# Autodesk Inventor assembly: tortoise
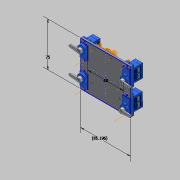
[picture p0: Inventor's stored thumbnail of the model, 180x180]
Saved by Autodesk Inventor 2014 SP2 (Build 180246200, 246)
## iProperties
Created: 2015-01-06
Part Number: tortoise
Document SubType Name: Assembly
Designer: lmarshall
Author: lmarshall
## Documents named in this file (4)
- C:\Users\lmarshall\Documents\tortoise\tortoise.iam
- C:\Users\lmarshall\Documents\tortoise\Base.ipt
- C:\Users\Public\Documents\Autodesk\Inventor 2014\Interactive Tutorial\Imported Components\SG90\SG90.iam
- C:\Users\Public\Documents\Autodesk\Inventor 2014\Interactive Tutorial\Imported Components\arduino uno\arduino uno.iam
## Components (6 placed, 3 different names)
1. Base:1 — Mate:1, Mate:3, Mate:4, Mate:7, Mate:8, Mate:9, Mate:11, Mate:12, Mate:13, Mate:16, Mate:17, Mate:23, Mate:24, Mate:27
2. SG90:1 [sub-assembly] — Mate:1, Mate:2, Mate:5
3. SG90:2 [sub-assembly] — Mate:7, Mate:10
4. SG90:3 [sub-assembly] — Mate:8, Mate:14, Mate:19
5. SG90:4 [sub-assembly] — Mate:9, Mate:15, Mate:21
6. arduino uno:1 [sub-assembly] — Mate:23, Mate:25, Mate:26
## Relationships (29: Mate 29)
- Mate:1: Base:1 ↔ SG90:1
- Mate:2: SG90:1
- Mate:3: Base:1
- Mate:4: Base:1
- Mate:5: SG90:1
- Mate:6
- Mate:7: Base:1 ↔ SG90:2
- Mate:8: Base:1 ↔ SG90:3
- Mate:9: Base:1 ↔ SG90:4
- Mate:10: SG90:2
- Mate:11: Base:1
- Mate:12: Base:1
- Mate:13: Base:1
- Mate:14: SG90:3
- Mate:15: SG90:4
- Mate:16: Base:1
- Mate:17: Base:1
- Mate:18
- Mate:19: SG90:3
- Mate:20
- Mate:21: SG90:4
- Mate:22
- Mate:23 (3 mm): Base:1 ↔ arduino uno:1
- Mate:24: Base:1
- Mate:25: arduino uno:1
- Mate:26: arduino uno:1
- Mate:27: Base:1
- Mate:28
- Mate:29
